# Autodesk Inventor assembly: Assembly5
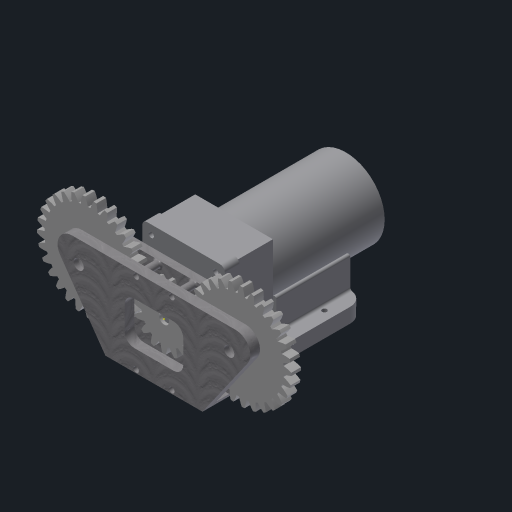
[picture p0: Inventor's stored thumbnail of the model, 512x512]
Saved by Autodesk Inventor 2024.3 (Build 283343000, 343)
## iProperties
Created: 2024-06-30
Part Number: Assembly5
Material: Generic
Document SubType Name: Assembly
Designer: Niler
Author: Niler
## Documents named in this file (4)
- C:\Users\Niler\OneDrive\Escritorio\RECICLADOR\RECICLADOR_MODELO_3D\CAJA_ENGRANAJES\VERSION_2\Assembly5 - Copy.iam
- C:\Users\Niler\OneDrive\Escritorio\RECICLADOR\RECICLADOR_MODELO_3D\MECANISMO DE COMPACTADO\SOPORTE DEL MOTOR.ipt
- C:\Users\Niler\OneDrive\Escritorio\RECICLADOR\RECICLADOR_MODELO_3D\MECANISMO DE COMPACTADO\MOTOR DC.ipt
- C:\Users\Niler\OneDrive\Escritorio\RECICLADOR\RECICLADOR_MODELO_3D\CAJA_ENGRANAJES\CAJA_ENGRANAJES_COMPLETA.iam
## Components (3 placed, 3 different names)
1. SOPORTE DEL MOTOR:1 — Angle:1, Mate:4, Mate:6, Mate:7, Mate:8
2. MOTOR DC:1 — Angle:1, Mate:4, Mate:5, Mate:6
3. CAJA_ENGRANAJES_COMPLETA:1 [sub-assembly] — Mate:5, Mate:7, Mate:8
## Relationships (6: Mate 5, Angle 1)
- Angle:1 (0 deg): SOPORTE DEL MOTOR:1 ↔ MOTOR DC:1
- Mate:4: SOPORTE DEL MOTOR:1 ↔ MOTOR DC:1
- Mate:5: MOTOR DC:1 ↔ CAJA_ENGRANAJES_COMPLETA:1
- Mate:6: SOPORTE DEL MOTOR:1 ↔ MOTOR DC:1
- Mate:7: SOPORTE DEL MOTOR:1 ↔ CAJA_ENGRANAJES_COMPLETA:1
- Mate:8: SOPORTE DEL MOTOR:1 ↔ CAJA_ENGRANAJES_COMPLETA:1
